# Autodesk Inventor assembly: One Character Step
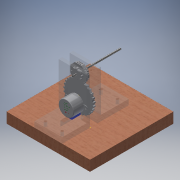
[picture p0: Inventor's stored thumbnail of the model, 180x180]
Saved by Autodesk Inventor 2017 (Build 210142000, 142)
## iProperties
Created: 2018-03-09
Part Number: One Character Step
Document SubType Name: Assembly
Designer: Russ
Author: Russ
## Documents named in this file (10)
- C:\Users\Russ\Desktop\3D Models\ORBD\One Character Step.iam
- C:\Users\Russ\Desktop\3D Models\ORBD\Base.ipt
- C:\Users\Russ\Desktop\3D Models\ORBD\Stepper Motor\5V DC STEP MOTOR.ipt
- C:\Users\Russ\Desktop\3D Models\ORBD\Stepper Motor Frame.ipt
- C:\Users\Russ\Desktop\3D Models\ORBD\Axle.ipt
- C:\Users\Russ\Desktop\3D Models\ORBD\8 ul Left Braille Wheel (Octagon).ipt
- C:\Users\Russ\Desktop\3D Models\ORBD\8 ul Right Braille Wheel (Nonagon).ipt
- C:\Users\Russ\Desktop\3D Models\ORBD\Hybrid Driver Gear.ipt
- C:\Users\Russ\Desktop\3D Models\ORBD\Middle Gear Frame.ipt
- C:\Users\Russ\Desktop\3D Models\ORBD\10 ul Middle Gear.ipt
## Components (9 placed, 9 different names)
1. Base:1 — Flush:1, Mate:4, Flush:2
2. 5V DC STEP MOTOR:1 — Mate:5, Mate:6, Flush:3, Mate:11, Mate:12
3. Stepper Motor Frame:1 — Flush:1, Mate:4, Flush:2, Mate:5, Mate:6, Flush:3, Mate:7, Flush:4, Angle:1, Mate:17
4. Axle:1 — Mate:7, Flush:4, Mate:8, Mate:9, Mate:13
5. 8 ul Left Braille Wheel (Octagon):1 — Mate:8, Mate:10, Mate:17, Rotation:3
6. 8 ul Right Braille Wheel (Nonagon):1 — Mate:9, Mate:10, Mate:16, Rotation:2
7. Hybrid Driver Gear:1 — Mate:11, Mate:12, Rotation:1, Rotation:3
8. Middle Gear Frame:1 — Mate:13, Angle:1, Mate:14, Mate:15, Mate:16
9. 10 ul Middle Gear:1 — Mate:14, Mate:15, Rotation:1, Rotation:2
## Relationships (22: Mate 14, Flush 4, RelateRotation 3, Angle 1)
- Flush:1: Base:1 ↔ Stepper Motor Frame:1
- Mate:4: Base:1 ↔ Stepper Motor Frame:1
- Flush:2 (-50.8 mm): Base:1 ↔ Stepper Motor Frame:1
- Mate:5: 5V DC STEP MOTOR:1 ↔ Stepper Motor Frame:1
- Mate:6: 5V DC STEP MOTOR:1 ↔ Stepper Motor Frame:1
- Flush:3 (18.1 mm): 5V DC STEP MOTOR:1 ↔ Stepper Motor Frame:1
- Mate:7: Stepper Motor Frame:1 ↔ Axle:1
- Flush:4: Stepper Motor Frame:1 ↔ Axle:1
- Mate:8: Axle:1 ↔ 8 ul Left Braille Wheel (Octagon):1
- Mate:9: Axle:1 ↔ 8 ul Right Braille Wheel (Nonagon):1
- Mate:10: 8 ul Left Braille Wheel (Octagon):1 ↔ 8 ul Right Braille Wheel (Nonagon):1
- Mate:11: 5V DC STEP MOTOR:1 ↔ Hybrid Driver Gear:1
- Mate:12: 5V DC STEP MOTOR:1 ↔ Hybrid Driver Gear:1
- Mate:13: Axle:1 ↔ Middle Gear Frame:1
- Angle:1 (0 deg): Stepper Motor Frame:1 ↔ Middle Gear Frame:1
- Mate:14: Middle Gear Frame:1 ↔ 10 ul Middle Gear:1
- Mate:15: Middle Gear Frame:1 ↔ 10 ul Middle Gear:1
- Mate:16: 8 ul Right Braille Wheel (Nonagon):1 ↔ Middle Gear Frame:1
- Mate:17: Stepper Motor Frame:1 ↔ 8 ul Left Braille Wheel (Octagon):1
- Rotation:1 [RelateRotation] (1 ul): Hybrid Driver Gear:1 ↔ 10 ul Middle Gear:1
- Rotation:2 [RelateRotation] (1 ul): 8 ul Right Braille Wheel (Nonagon):1 ↔ 10 ul Middle Gear:1
- Rotation:3 [RelateRotation] (3.375 ul): 8 ul Left Braille Wheel (Octagon):1 ↔ Hybrid Driver Gear:1
